# Autodesk Inventor assembly: ELP Camera
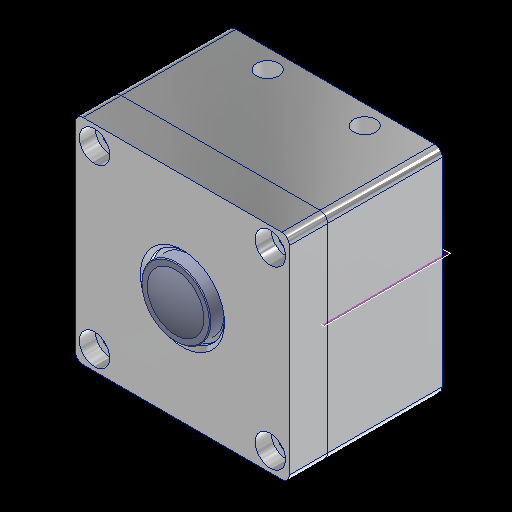
[picture p0: Inventor's stored thumbnail of the model, 512x512]
Saved by Autodesk Inventor 2023.3 (Build 273359000, 359)
## iProperties
Created: 2024-02-12
Part Number: ELP Camera
Document SubType Name: Assembly
Designer: mavericks
Mass: 119.364 g
Surface Area: 380.418 cm^2
Volume: 44.209 cm^3
Density: 2.7 g/cm^3
Author: mavericks
## Documents named in this file (4)
- C:\Users\mavericks\Desktop\Crescendo_2024-CAD\2024 Robot\COMMON PARTS\ELECTRONICS\cameras\ELP Camera.iam
- C:\Users\mavericks\Desktop\Crescendo_2024-CAD\2024 Robot\COMMON PARTS\ELECTRONICS\cameras\ELP Camera Case.ipt
- C:\Users\mavericks\Desktop\Crescendo_2024-CAD\2024 Robot\COMMON PARTS\ELECTRONICS\cameras\ELP Camera.ipt
- C:\Users\mavericks\Desktop\Crescendo_2024-CAD\2024 Robot\COMMON PARTS\ELECTRONICS\cameras\ELP Camera Lid.ipt
## Components (3 placed, 3 different names)
1. ELP Camera Case:1 — Insert:1, Mate:1, Insert:2, Insert:3, Insert:4, Insert:5
2. ELP Camera:1 — Insert:1, Mate:1
3. ELP Camera Lid:1 — Insert:2, Insert:3, Insert:4, Insert:5
## Relationships (6: Insert 5, Mate 1)
- Insert:1: ELP Camera Case:1 ↔ ELP Camera:1
- Mate:1: ELP Camera Case:1 ↔ ELP Camera:1
- Insert:2: ELP Camera Case:1 ↔ ELP Camera Lid:1
- Insert:3: ELP Camera Case:1 ↔ ELP Camera Lid:1
- Insert:4: ELP Camera Case:1 ↔ ELP Camera Lid:1
- Insert:5: ELP Camera Case:1 ↔ ELP Camera Lid:1
